# Autodesk Inventor assembly: skipper
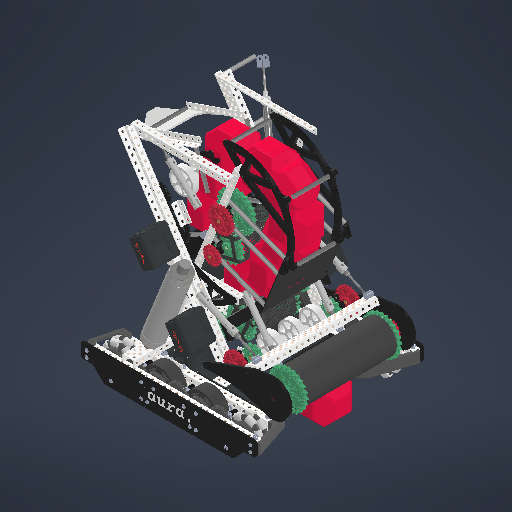
[picture p0: Inventor's stored thumbnail of the model, 512x512]
Saved by Autodesk Inventor 2025.2 (Build 292293000, 293)
## iProperties
Created: 2026-01-02
Part Number: skipper
Document SubType Name: Assembly
Designer: cloudy
Author: cloudy
## Documents named in this file (14)
- C:\Users\cloudy\Documents\GitHub\aura-cad\24\skipper.iam
- C:\Users\cloudy\Documents\GitHub\aura-cad\24\Drivetrain\!drivetrain.iam
- C:\Users\cloudy\Documents\GitHub\aura-cad\24\structure.iam
- C:\Users\cloudy\Documents\GitHub\aura-cad\15\25 stroke 10 bore\CJ2D10-25Z(0_0).iam
- C:\Users\cloudy\Documents\GitHub\aura-cad\24\intakeside.ipt
- C:\Users\cloudy\Documents\GitHub\aura-cad\!lib\Structure\C Channel\Aluminum 1x3x1 Half\Alu C Half 1x3x1x2.ipt
- C:\Users\cloudy\Documents\GitHub\aura-cad\!lib\Structure\C Channel\Aluminum 1x2x1\Alu C 1x2x1x20.ipt
- C:\Users\cloudy\Documents\GitHub\aura-cad\!lib\Motion\Shaft LS\Shaft Collar Metal\Shaft Collar No Screw.iam
- C:\Users\cloudy\Documents\AURA_CAD\!lib\Motion\Shaft LS\Shaft Collar Metal.iam
- C:\Users\cloudy\Documents\GitHub\aura-cad\24\bottom rails.ipt
- C:\Users\cloudy\Documents\GitHub\aura-cad\!lib\Structure\Standoff\Standoff 5.00.ipt
- C:\Users\cloudy\Documents\AURA_CAD\!lib\Structure\Standoff.ipt
- C:\Users\cloudy\Documents\GitHub\aura-cad\!lib\Structure\Standoff\Standoff 3.00.ipt
- C:\Users\cloudy\Documents\GitHub\aura-cad\!lib\Miscellaneous\iw_metal_02.bmp
## Components (23 placed, 10 different names)
1. !drivetrain:1 [sub-assembly] — Insert:1, Mate:1
2. structure:1 [sub-assembly] — Insert:1, Mate:1, Insert:2, Insert:3, Mate:3, Mate:7, Mate:8, Insert:14, Mate:9, Insert:15, Insert:16, Insert:17
3. intakeside:1 — Insert:2, Mate:2, Mate:3, Insert:4, Mate:4
4. intakeside:2 — Insert:3, Mate:2, Insert:5, Mate:5
5. Alu C Half 1x3x1x2:1 — Insert:4, Mate:4, Insert:6, Mate:6
6. Alu C Half 1x3x1x2:2 — Insert:5, Mate:5
7. Alu C 1x2x1x20:1 — Insert:6, Mate:6, Insert:10, Insert:13
8. CJ2D10-25Z(0_0):1 [sub-assembly] — Insert:9, Mate:7
9. Shaft Collar No Screw:1 [sub-assembly] — Insert:8, Insert:10
10. Shaft Collar No Screw:2 [sub-assembly] — Insert:8, Insert:9
11. CJ2D10-25Z(0_0):2 [sub-assembly] — Mate:8
12. Shaft Collar No Screw:3 [sub-assembly] — Insert:13
13. Shaft Collar No Screw:4 [sub-assembly]
14. bottom rails:1 — Insert:14, Mate:9, Insert:18, Insert:19, Insert:20, Insert:21, Insert:22, Insert:23
15. Standoff 5.00:1 — Insert:21
16. Standoff 5.00:2 — Insert:20
17. Standoff 5.00:3 — Insert:18
18. Standoff 5.00:4 — Insert:19
19. Standoff 3.00:5 — Insert:15
20. Standoff 3.00:6 — Insert:17
21. Standoff 3.00:7 — Insert:16
22. Standoff 5.00:8 — Insert:23
23. Standoff 5.00:9 — Insert:22
## Relationships (31: Insert 22, Mate 9)
- Insert:1 (3.175 mm): !drivetrain:1 ↔ structure:1
- Mate:1: !drivetrain:1 ↔ structure:1
- Insert:2 (31.75 mm): structure:1 ↔ intakeside:1
- Insert:3 (31.75 mm): structure:1 ↔ intakeside:2
- Mate:2: intakeside:1 ↔ intakeside:2
- Mate:3: structure:1 ↔ intakeside:1
- Insert:4: intakeside:1 ↔ Alu C Half 1x3x1x2:1
- Mate:4: intakeside:1 ↔ Alu C Half 1x3x1x2:1
- Insert:5: intakeside:2 ↔ Alu C Half 1x3x1x2:2
- Mate:5: intakeside:2 ↔ Alu C Half 1x3x1x2:2
- Insert:6: Alu C Half 1x3x1x2:1 ↔ Alu C 1x2x1x20:1
- Mate:6: Alu C Half 1x3x1x2:1 ↔ Alu C 1x2x1x20:1
- Insert:8: Shaft Collar No Screw:1 ↔ Shaft Collar No Screw:2
- Insert:9 (-2.54 mm): CJ2D10-25Z(0_0):1 ↔ Shaft Collar No Screw:2
- Insert:10: Alu C 1x2x1x20:1 ↔ Shaft Collar No Screw:1
- Mate:7: structure:1 ↔ CJ2D10-25Z(0_0):1
- [Insert]: Shaft Collar No Screw:3 ↔ Shaft Collar No Screw:4
- [Insert] (-2.54 mm): CJ2D10-25Z(0_0):2 ↔ Shaft Collar No Screw:4
- Insert:13: Alu C 1x2x1x20:1 ↔ Shaft Collar No Screw:3
- Mate:8: structure:1 ↔ CJ2D10-25Z(0_0):2
- Insert:14 (120.65 mm): structure:1 ↔ bottom rails:1
- Mate:9: structure:1 ↔ bottom rails:1
- Insert:15 (7.9375 mm): structure:1 ↔ Standoff 3.00:5
- Insert:16 (7.9375 mm): structure:1 ↔ Standoff 3.00:7
- Insert:17 (7.9375 mm): structure:1 ↔ Standoff 3.00:6
- Insert:18: bottom rails:1 ↔ Standoff 5.00:3
- Insert:19: bottom rails:1 ↔ Standoff 5.00:4
- Insert:20: bottom rails:1 ↔ Standoff 5.00:2
- Insert:21: bottom rails:1 ↔ Standoff 5.00:1
- Insert:22: bottom rails:1 ↔ Standoff 5.00:9
- Insert:23: bottom rails:1 ↔ Standoff 5.00:8
## Named parameters: d21_d16 = 0 mm, d22_d17 = -2.54 mm
